# Autodesk Inventor assembly: chassis
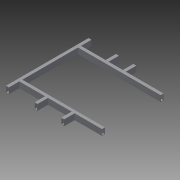
[picture p0: Inventor's stored thumbnail of the model, 180x180]
Saved by Autodesk Inventor 2015 (Build 190159000, 159)
## iProperties
Created: 2016-01-16
Part Number: chassis
Document SubType Name: Assembly
Designer: gus
Author: gus
## Documents named in this file (3)
- \\Mac\Google Drive\2016 Robot CAD\chassis.iam
- \\Mac\Google Drive\2016 Robot CAD\1x2x28.ipt
- \\Mac\Google Drive\2016 Robot CAD\1X2- bumper support.ipt
## Components (7 placed, 2 different names)
1. 1x2x28:1 — Mate:1, Flush:1, Mate:2, Flush:2, Flush:5, Flush:8
2. 1x2x28:2 — Mate:2, Flush:2, Mate:5, Mate:6, Flush:6, Flush:7
3. 1x2x28:3 — Mate:1, Flush:1, Mate:3, Mate:4, Flush:3, Flush:4
4. 1X2- bumper support:1 — Mate:5, Flush:7, Flush:8
5. 1X2- bumper support:2 — Mate:3, Flush:3, Flush:5
6. 1X2- bumper support:3 — Mate:6, Flush:6
7. 1X2- bumper support:4 — Mate:4, Flush:4
## Relationships (14: Flush 8, Mate 6)
- Mate:1: 1x2x28:1 ↔ 1x2x28:3
- Flush:1: 1x2x28:1 ↔ 1x2x28:3
- Mate:2: 1x2x28:1 ↔ 1x2x28:2
- Flush:2: 1x2x28:1 ↔ 1x2x28:2
- Mate:3: 1x2x28:3 ↔ 1X2- bumper support:2
- Mate:4: 1x2x28:3 ↔ 1X2- bumper support:4
- Flush:3: 1x2x28:3 ↔ 1X2- bumper support:2
- Flush:4: 1x2x28:3 ↔ 1X2- bumper support:4
- Flush:5: 1x2x28:1 ↔ 1X2- bumper support:2
- Mate:5: 1x2x28:2 ↔ 1X2- bumper support:1
- Mate:6: 1x2x28:2 ↔ 1X2- bumper support:3
- Flush:6: 1x2x28:2 ↔ 1X2- bumper support:3
- Flush:7: 1x2x28:2 ↔ 1X2- bumper support:1
- Flush:8: 1x2x28:1 ↔ 1X2- bumper support:1
